# Autodesk Inventor assembly: Assembly3
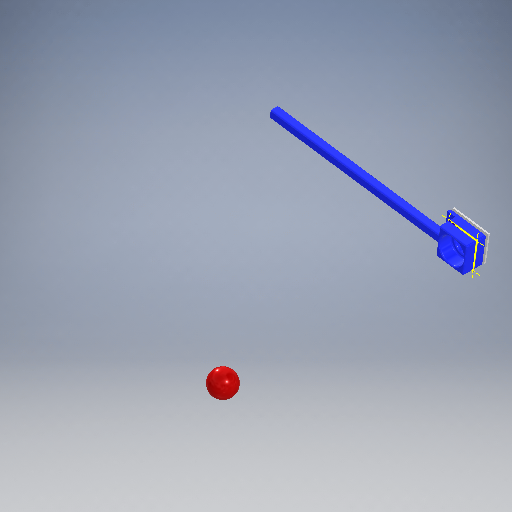
[picture p0: Inventor's stored thumbnail of the model, 512x512]
Saved by Autodesk Inventor 2025.3 (Build 293356000, 356)
## iProperties
Created: 2026-03-06
Part Number: Assembly3
Document SubType Name: Assembly
Designer: user
Author: user
## Documents named in this file (4)
- C:\Ayman\Inventor Projects\Lifting Mechanism\Assembly3.iam
- C:\Ayman\Inventor Projects\Lifting Mechanism\arm.ipt
- C:\Ayman\Inventor Projects\Lifting Mechanism\sensor.ipt
- C:\Ayman\Inventor Projects\Lifting Mechanism\ball.ipt
## Components (3 placed, 3 different names)
1. arm:1 — Mate:1, Mate:2, Mate:3, Mate:4, Mate:5
2. sensor:1 — Mate:1, Mate:2, Mate:3, Mate:4
3. ball:1 — Mate:5
## Relationships (5: Mate 5)
- Mate:1: arm:1 ↔ sensor:1
- Mate:2: arm:1 ↔ sensor:1
- Mate:3: arm:1 ↔ sensor:1
- Mate:4: arm:1 ↔ sensor:1
- Mate:5: arm:1 ↔ ball:1
